# Autodesk Inventor assembly: 489 Forest
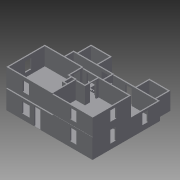
[picture p0: Inventor's stored thumbnail of the model, 180x180]
Saved by Autodesk Inventor 2013 SP2 (Build 170200200, 200)
## iProperties
Created: 2014-06-02
Part Number: 489 Forest
Document SubType Name: Assembly
Designer: jmw3
Author: jmw3
## Documents named in this file (3)
- F:\NIST\House Drawings\489 Forest.iam
- F:\NIST\House Drawings\489 Forest 1st Floor.ipt
- F:\NIST\House Drawings\489 Forest 2nd Floor.ipt
## Components (2 placed, 2 different names)
1. 489 Forest 1st Floor:1 — Flush:1, Mate:1, Flush:2, Flush:3, Mate:2, Flush:4
2. 489 Forest 2nd Floor:1 — Flush:1, Mate:1, Flush:2, Flush:3, Mate:2, Flush:4
## Relationships (6: Flush 4, Mate 2)
- Flush:1: 489 Forest 1st Floor:1 ↔ 489 Forest 2nd Floor:1
- Mate:1: 489 Forest 1st Floor:1 ↔ 489 Forest 2nd Floor:1
- Flush:2: 489 Forest 1st Floor:1 ↔ 489 Forest 2nd Floor:1
- Flush:3: 489 Forest 1st Floor:1 ↔ 489 Forest 2nd Floor:1
- Mate:2: 489 Forest 1st Floor:1 ↔ 489 Forest 2nd Floor:1
- Flush:4: 489 Forest 1st Floor:1 ↔ 489 Forest 2nd Floor:1
